# Autodesk Inventor assembly: ServoBlockLargeServoPlate
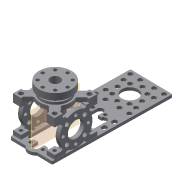
[picture p0: Inventor's stored thumbnail of the model, 180x180]
Saved by Autodesk Inventor 2018 (Build 220112000, 112)
## iProperties
Created: 2018-10-26
Part Number: ServoBlockLargeServoPlate
Document SubType Name: Assembly
Designer: ball
Author: ball
## Documents named in this file (5)
- C:\FTC\FTC8863CAD\2018Robot\ServoBlockLargeServoPlate.iam
- C:\FTC\FTC8863CAD\Actobotics\637 parts\637112\535118 assembly.ipt
- C:\FTC\FTC8863CAD\Actobotics\637 parts\637112\525123.ipt
- C:\FTC\FTC8863CAD\Actobotics\637 parts\637112\545420.ipt
- C:\FTC\FTC8863CAD\Actobotics\575 parts\575144.ipt
## Components (5 placed, 4 different names)
1. 535118 assembly:1 — Mate:8, Mate:9, Mate:10, Mate:11
2. 525123:1 — Mate:11, Mate:12
3. 545420:1 — Mate:1, Mate:2, Mate:3, Mate:8, Mate:9, Symmetry:1
4. 545420:2 — Mate:4, Mate:5, Mate:6, Mate:10, Symmetry:1
5. 575144:1 — Mate:1, Mate:2, Mate:3, Mate:4, Mate:5, Mate:6, Mate:12
## Relationships (12: Mate 11, Symmetry 1)
- Mate:1: 545420:1 ↔ 575144:1
- Mate:2: 545420:1 ↔ 575144:1
- Mate:3: 545420:1 ↔ 575144:1
- Mate:4: 545420:2 ↔ 575144:1
- Mate:5: 545420:2 ↔ 575144:1
- Mate:6: 545420:2 ↔ 575144:1
- Mate:8: 535118 assembly:1 ↔ 545420:1
- Mate:9: 535118 assembly:1 ↔ 545420:1
- Mate:10: 535118 assembly:1 ↔ 545420:2
- Mate:11: 535118 assembly:1 ↔ 525123:1
- Mate:12 (12.4968 mm): 525123:1 ↔ 575144:1
- Symmetry:1: 545420:1 ↔ 545420:2
